# Autodesk Inventor assembly: мёртвое колесо_MIR6_MIR_MIR1_MIR
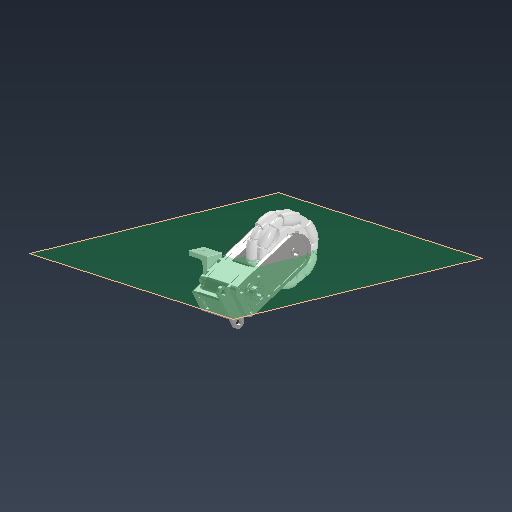
[picture p0: Inventor's stored thumbnail of the model, 512x512]
Saved by Autodesk Inventor 2025 (Build 290162000, 162)
## iProperties
Created: 2024-08-28
Part Number: мёртвое колесо_MIR6_MIR_MIR1_MIR
Document SubType Name: Assembly
Designer: GameHD
Author: Phantom
## Documents named in this file (7)
- C:\Users\GameHD\Desktop\Phantom 16950\мёртвое колесо_MIR6_MIR_MIR1_MIR.iam
- C:\Users\GameHD\Desktop\Phantom 16950\3110-0001-0001 assembly_MIR4_MIR_MIR1_MIR.iam
- C:\Users\GameHD\Desktop\Phantom 16950\1120-0003-0096_MIR1_MIR4_MIR_MIR1_MIR.ipt
- C:\Users\GameHD\Desktop\Phantom 16950\2915-0001-0003\2915-0001-0003_MIR2_MIR_MIR1_MIR.ipt
- C:\Users\GameHD\Desktop\Phantom 16950\1502-0006-0120\1502-0006-0120_MIR2_MIR_MIR1_MIR.ipt
- C:\Users\GameHD\Desktop\Phantom 16950\2800-0004-0020\2800-0004-0020_MIR2_MIR_MIR1_MIR.ipt
- C:\Users\GameHD\Desktop\Phantom 16950\2812-0004-0007\2812-0004-0007_MIR2_MIR_MIR1_MIR.ipt
## Components (6 placed, 6 different names)
1. 3110-0001-0001 assembly_MIR4_MIR_MIR1_MIR:1 [sub-assembly] — Совмещение:5
2. 1120-0003-0096_MIR1_MIR4_MIR_MIR1_MIR:1 — Совмещение:5, Заподлицо:1
3. 2915-0001-0003_MIR2_MIR_MIR1_MIR:1
4. 1502-0006-0120_MIR2_MIR_MIR1_MIR:1 — Совмещение:4
5. 2800-0004-0020_MIR2_MIR_MIR1_MIR:1 — Совмещение:4, Совмещение:5
6. 2812-0004-0007_MIR2_MIR_MIR1_MIR:1 — Совмещение:5
## Relationships (4: Mate 3, Flush 1)
- Совмещение:5 [Mate]: 3110-0001-0001 assembly_MIR4_MIR_MIR1_MIR:1 ↔ 1120-0003-0096_MIR1_MIR4_MIR_MIR1_MIR:1
- Совмещение:4 [Mate]: 1502-0006-0120_MIR2_MIR_MIR1_MIR:1 ↔ 2800-0004-0020_MIR2_MIR_MIR1_MIR:1
- Совмещение:5 [Mate]: 2800-0004-0020_MIR2_MIR_MIR1_MIR:1 ↔ 2812-0004-0007_MIR2_MIR_MIR1_MIR:1
- Заподлицо:1 [Flush]: 1120-0003-0096_MIR1_MIR4_MIR_MIR1_MIR:1
